# Autodesk Inventor assembly: Base
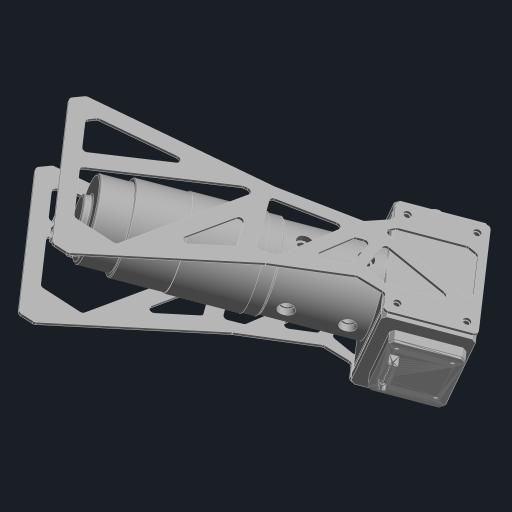
[picture p0: Inventor's stored thumbnail of the model, 512x512]
Saved by Autodesk Inventor 2023 (Build 270158000, 158)
## iProperties
Created: 2020-03-24
Part Number: Base
Document SubType Name: Assembly
Designer: valer
Mass: 715.256 g
Surface Area: 821.775 cm^2
Volume: 200.817 cm^3
Density: 3.56173 g/cm^3
Author: valer
## Documents named in this file (8)
- C:\Users\valer\Desktop\str1ker\cad\ArmBase.iam
- C:\Users\valer\Desktop\str1ker\cad\external\ShoulderActuator\DumaDynamics00E.ipt
- C:\Users\valer\Desktop\str1ker\cad\ShoulderMotorMount.ipt
- C:\Users\valer\Desktop\str1ker\cad\ShoulderEncoderSpacer.ipt
- C:\Users\valer\Desktop\str1ker\cad\external\ShoulderEncoder\ArmEncoderBoard.ipt
- C:\Users\valer\Desktop\str1ker\cad\ShoulderMount.ipt
- C:\Users\valer\Desktop\str1ker\cad\external\ArmEncoder\ArmEncoderShaftMagnet6mm.ipt
- C:\Users\valer\Desktop\str1ker\cad\ArmBaseEncoderAlignmentFlange.ipt
## Components (9 placed, 7 different names)
1. DumaDynamics00E:1 — Mate:1, Flush:1, Mate:2, Mate:3, Mate:4, Mate:16, Mate:17, Mate:19
2. ShoulderMotorMount:1 — Mate:1, Mate:2, Mate:3, Flush:2, Mate:5, Mate:6, Mate:15, Flush:3, Mate:22, Mate:23, Mate:24
3. ShoulderMotorMount:2 — Mate:4, Mate:5, Mate:6, Mate:9, Mate:10, Mate:11, Mate:20
4. ShoulderEncoderSpacer:1 — Mate:9, Mate:10, Mate:11, Mate:14
5. ArmEncoderBoard:1 — Mate:14, Mate:20, Mate:21
6. ShoulderMount:1 — Flush:3
7. ArmEncoderShaftMagnet6mm:1 — Mate:16, Mate:17, Mate:18, Mate:21
8. ArmBaseEncoderAlignmentFlange:1 — Mate:18, Mate:19
9. ShoulderMount:2 — Mate:22, Mate:23, Mate:24
## Relationships (23: Mate 20, Flush 3)
- Mate:1: DumaDynamics00E:1 ↔ ShoulderMotorMount:1
- Flush:1: DumaDynamics00E:1
- Mate:2: DumaDynamics00E:1 ↔ ShoulderMotorMount:1
- Mate:3: DumaDynamics00E:1 ↔ ShoulderMotorMount:1
- Flush:2: ShoulderMotorMount:1
- Mate:4: DumaDynamics00E:1 ↔ ShoulderMotorMount:2
- Mate:5: ShoulderMotorMount:1 ↔ ShoulderMotorMount:2
- Mate:6: ShoulderMotorMount:1 ↔ ShoulderMotorMount:2
- Mate:9: ShoulderMotorMount:2 ↔ ShoulderEncoderSpacer:1
- Mate:10: ShoulderMotorMount:2 ↔ ShoulderEncoderSpacer:1
- Mate:11: ShoulderMotorMount:2 ↔ ShoulderEncoderSpacer:1
- Mate:14: ShoulderEncoderSpacer:1 ↔ ArmEncoderBoard:1
- Mate:15: ShoulderMotorMount:1
- Flush:3: ShoulderMotorMount:1 ↔ ShoulderMount:1
- Mate:16: DumaDynamics00E:1 ↔ ArmEncoderShaftMagnet6mm:1
- Mate:17: DumaDynamics00E:1 ↔ ArmEncoderShaftMagnet6mm:1
- Mate:18: ArmEncoderShaftMagnet6mm:1 ↔ ArmBaseEncoderAlignmentFlange:1
- Mate:19: DumaDynamics00E:1 ↔ ArmBaseEncoderAlignmentFlange:1
- Mate:20: ShoulderMotorMount:2 ↔ ArmEncoderBoard:1
- Mate:21 (0.3 mm): ArmEncoderBoard:1 ↔ ArmEncoderShaftMagnet6mm:1
- Mate:22: ShoulderMotorMount:1 ↔ ShoulderMount:2
- Mate:23: ShoulderMotorMount:1 ↔ ShoulderMount:2
- Mate:24: ShoulderMotorMount:1 ↔ ShoulderMount:2
